# Autodesk Inventor assembly: Main-Bot-Assembly-Version-2
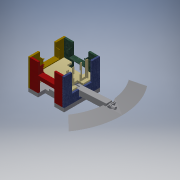
[picture p0: Inventor's stored thumbnail of the model, 180x180]
Saved by Autodesk Inventor 2017.3 (Build 213256000, 256)
## iProperties
Created: 2018-03-05
Part Number: Main-Bot-Assembly-Version-2
Document SubType Name: Assembly
Designer: Harsh Gupta
Sending System: Autodesk Inventor 2018
Preprocessor: ST-DEVELOPER v16.13
Title: C:\Users\harsh\Documents\Inventor\BigMac Sumobot\Main Bot Assembly Version 2.stp
Author: harsh
## Documents named in this file (17)
- C:\Users\Jeff Suitor\Desktop\Main Bot Print Ready\Main-Bot-Assembly-Version-2.iam
- C:\Users\Jeff Suitor\Desktop\Main Bot Print Ready\Body Base Plate.ipt
- C:\Users\Jeff Suitor\Desktop\Main Bot Print Ready\HC-SR04.ipt
- C:\Users\Jeff Suitor\Desktop\Main Bot Print Ready\HC-SR04_MIR.ipt
- C:\Users\Jeff Suitor\Desktop\Main Bot Print Ready\HC-SR04_MIR1.ipt
- C:\Users\Jeff Suitor\Desktop\Main Bot Print Ready\Arduino_Uno.ipt
- C:\Users\Jeff Suitor\Desktop\Main Bot Print Ready\42x19 Wheel.ipt
- C:\Users\Jeff Suitor\Desktop\Main Bot Print Ready\Motor.ipt
- C:\Users\Jeff Suitor\Desktop\Main Bot Print Ready\Bottom Base Plate.ipt
- C:\Users\Jeff Suitor\Desktop\Main Bot Print Ready\Reflectance Sensor.ipt
- C:\Users\Jeff Suitor\Desktop\Main Bot Print Ready\Back Plate V3.ipt
- C:\Users\Jeff Suitor\Desktop\Main Bot Print Ready\Front Plate V3.ipt
- C:\Users\Jeff Suitor\Desktop\Main Bot Print Ready\Side Panels V2.ipt
- C:\Users\Jeff Suitor\Desktop\Main Bot Print Ready\Paddle Assembly.iam
- C:\Users\Jeff Suitor\Desktop\Main Bot Print Ready\Peddal Left.ipt
- C:\Users\Jeff Suitor\Desktop\Main Bot Print Ready\Peddal Right.ipt
- C:\Users\Jeff Suitor\Desktop\Main Bot Print Ready\Nut.ipt
## Components (24 placed, 17 different names)
1. Body Base Plate:1 — Mate:1, Mate:2, Mate:3, Mate:4, Mate:5, Flush:4, Flush:5, Flush:6, Mate:17, Flush:19, Flush:20, Mate:21, Mate:29, Flush:32
2. HC-SR04:3 — Flush:17, Flush:20, Flush:21, Mate:21
3. HC-SR04:6 — Flush:2, Mate:3, Mate:4
4. HC-SR04_MIR:2 — Flush:1, Mate:1, Mate:2, Flush:27
5. HC-SR04_MIR1:1 — Flush:18, Flush:19, Flush:21
6. HC-SR04_MIR1:2 — Mate:5, Flush:4, Flush:24, Flush:30
7. Arduino_Uno:1 — Mate:17, Flush:32
8. 42x19 Wheel:1 — Flush:1, Insert:1
9. 42x19 Wheel:2 — Flush:2, Insert:2
10. Motor:1 — Mate:7, Flush:7, Tangent:1, Insert:1
11. Motor:2 — Mate:8, Flush:8, Tangent:2, Insert:2
12. Bottom Base Plate:1 — Flush:5, Flush:6, Mate:7, Flush:7, Tangent:1, Mate:8, Flush:8, Tangent:2, Mate:9, Mate:10, Mate:11, Mate:12, Mate:13, Mate:14, Mate:15, Mate:16, Flush:15, Mate:20, Flush:16, Mate:22, Flush:22, Flush:23, Mate:25, Flush:26, Mate:27, Mate:28, Mate:29, Flush:28, Mate:32, Flush:29, Flush:33, Flush:34, Mate:38, Mate:39, Mate:40, Mate:41
13. Reflectance Sensor:1 — Mate:15, Mate:16, Mate:38
14. Reflectance Sensor:2 — Mate:9, Mate:10, Mate:39
15. Reflectance Sensor:3 — Mate:13, Mate:14, Mate:40
16. Reflectance Sensor:4 — Mate:11, Mate:12, Mate:41
17. Back Plate V3:2 — Flush:15, Mate:20, Flush:16, Flush:17, Flush:18
18. Front Plate V3:1 — Mate:22, Flush:22, Flush:23, Flush:24, Mate:26, Flush:30
19. Right Panel — Flush:28, Mate:32, Flush:29
20. Left Panel — Mate:25, Mate:26, Flush:26, Flush:27
21. Paddle Assembly:1 [sub-assembly] — Mate:27, Mate:28, Angle:1, Mate:34, Mate:35, Mate:36, Mate:37
22. Peddal Left:1 — Flush:31, Mate:33, Mate:34, Mate:35
23. Peddal Right:1 — Flush:31, Angle:1, Mate:33
24. Nut:1 — Mate:36, Mate:37
## Relationships (66: Mate 35, Flush 26, Tangent 2, Insert 2, Angle 1)
- Flush:1: HC-SR04_MIR:2 ↔ 42x19 Wheel:1
- Mate:1 (15 mm): Body Base Plate:1 ↔ HC-SR04_MIR:2
- Mate:2: Body Base Plate:1 ↔ HC-SR04_MIR:2
- Flush:2: HC-SR04:6 ↔ 42x19 Wheel:2
- Mate:3 (15 mm): Body Base Plate:1 ↔ HC-SR04:6
- Mate:4: Body Base Plate:1 ↔ HC-SR04:6
- Mate:5 (15 mm): Body Base Plate:1 ↔ HC-SR04_MIR1:2
- Flush:4 (22.5 mm): Body Base Plate:1 ↔ HC-SR04_MIR1:2
- Flush:5 (5 mm): Body Base Plate:1 ↔ Bottom Base Plate:1
- Flush:6 (5 mm): Body Base Plate:1 ↔ Bottom Base Plate:1
- Mate:7: Motor:1 ↔ Bottom Base Plate:1
- Flush:7: Motor:1 ↔ Bottom Base Plate:1
- Tangent:1: Motor:1 ↔ Bottom Base Plate:1
- Insert:1 (-11 mm): 42x19 Wheel:1 ↔ Motor:1
- Mate:8: Motor:2 ↔ Bottom Base Plate:1
- Flush:8: Motor:2 ↔ Bottom Base Plate:1
- Tangent:2: Motor:2 ↔ Bottom Base Plate:1
- Insert:2 (-11 mm): 42x19 Wheel:2 ↔ Motor:2
- Mate:9: Bottom Base Plate:1 ↔ Reflectance Sensor:2
- Mate:10: Bottom Base Plate:1 ↔ Reflectance Sensor:2
- Mate:11: Bottom Base Plate:1 ↔ Reflectance Sensor:4
- Mate:12: Bottom Base Plate:1 ↔ Reflectance Sensor:4
- Mate:13: Bottom Base Plate:1 ↔ Reflectance Sensor:3
- Mate:14: Bottom Base Plate:1 ↔ Reflectance Sensor:3
- Mate:15: Bottom Base Plate:1 ↔ Reflectance Sensor:1
- Mate:16: Bottom Base Plate:1 ↔ Reflectance Sensor:1
- Mate:17: Body Base Plate:1 ↔ Arduino_Uno:1
- Flush:15: Bottom Base Plate:1 ↔ Back Plate V3:2
- Mate:20: Bottom Base Plate:1 ↔ Back Plate V3:2
- Flush:16: Bottom Base Plate:1 ↔ Back Plate V3:2
- Flush:17: HC-SR04:3 ↔ Back Plate V3:2
- Flush:18: HC-SR04_MIR1:1 ↔ Back Plate V3:2
- Flush:19 (17 mm): Body Base Plate:1 ↔ HC-SR04_MIR1:1
- Flush:20 (17 mm): Body Base Plate:1 ↔ HC-SR04:3
- Flush:21: HC-SR04:3 ↔ HC-SR04_MIR1:1
- Mate:21: Body Base Plate:1 ↔ HC-SR04:3
- Mate:22: Bottom Base Plate:1 ↔ Front Plate V3:1
- Flush:22: Bottom Base Plate:1 ↔ Front Plate V3:1
- Flush:23: Bottom Base Plate:1 ↔ Front Plate V3:1
- Flush:24: HC-SR04_MIR1:2 ↔ Front Plate V3:1
- Mate:25: Bottom Base Plate:1 ↔ Left Panel
- Mate:26: Front Plate V3:1 ↔ Left Panel
- Flush:26: Bottom Base Plate:1 ↔ Left Panel
- Mate:27: Bottom Base Plate:1 ↔ Paddle Assembly:1
- Mate:28: Bottom Base Plate:1 ↔ Paddle Assembly:1
- Mate:29 (23 mm): Body Base Plate:1 ↔ Bottom Base Plate:1
- [Mate]: Peddal Left:1 ↔ Peddal Right:1
- Flush:27: HC-SR04_MIR:2 ↔ Left Panel
- Flush:28: Bottom Base Plate:1 ↔ Right Panel
- Mate:32: Bottom Base Plate:1 ↔ Right Panel
- Flush:29 (5 mm): Bottom Base Plate:1 ↔ Right Panel
- Flush:30: HC-SR04_MIR1:2 ↔ Front Plate V3:1
- Flush:31: Peddal Left:1 ↔ Peddal Right:1
- Angle:1 (0 deg): Paddle Assembly:1 ↔ Peddal Right:1
- Flush:32: Body Base Plate:1 ↔ Arduino_Uno:1
- Mate:33: Peddal Left:1 ↔ Peddal Right:1
- Mate:34: Paddle Assembly:1 ↔ Peddal Left:1
- Mate:35: Paddle Assembly:1 ↔ Peddal Left:1
- Mate:36: Paddle Assembly:1 ↔ Nut:1
- Mate:37: Paddle Assembly:1 ↔ Nut:1
- Flush:33 (-30 mm): Bottom Base Plate:1
- Flush:34 (-50 mm): Bottom Base Plate:1
- Mate:38: Bottom Base Plate:1 ↔ Reflectance Sensor:1
- Mate:39: Bottom Base Plate:1 ↔ Reflectance Sensor:2
- Mate:40: Bottom Base Plate:1 ↔ Reflectance Sensor:3
- Mate:41: Bottom Base Plate:1 ↔ Reflectance Sensor:4
## Named parameters: d64_d1 = 0 mm
